# Autodesk Inventor assembly: ensamblaje jeringa
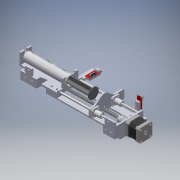
[picture p0: Inventor's stored thumbnail of the model, 180x180]
Saved by Autodesk Inventor 2019 (Build 230136000, 136)
## iProperties
Created: 2019-09-29
Part Number: ensamblaje jeringa
Document SubType Name: Assembly
Designer: dbrau
Author: dbrau
## Documents named in this file (13)
- D:\U\Semestre III mecánica\seminario\ensamblaje jeringa.iam
- D:\U\Semestre III mecánica\seminario\User Library-SYRINGE, MONOJECT, 60cc.ipt
- D:\U\Semestre III mecánica\seminario\sujeta_jeringa.ipt
- D:\U\Semestre III mecánica\seminario\NEMA 17 with T5 Pulley.iam
- D:\U\Semestre III mecánica\seminario\Acople flexible de aluminio (5mm a 8mm) Cimech 3D.ipt
- D:\U\Semestre III mecánica\seminario\Husillo Tr8x8 (p2) x 200mm real.ipt
- D:\U\Semestre III mecánica\seminario\LMK8UU.ipt
- D:\U\Semestre III mecánica\seminario\Tuerca Tr8x8 Cimech 3D.ipt
- D:\U\Semestre III mecánica\seminario\empuja_jeringa.ipt
- D:\U\Semestre III mecánica\seminario\sop_step_jeringa.ipt
- D:\U\Semestre III mecánica\seminario\eje_jeringa.ipt
- D:\U\Semestre III mecánica\seminario\union_jeringa.ipt
- D:\U\Semestre III mecánica\seminario\Endstop mecânico - Chave fim de curso.ipt
## Components (16 placed, 12 different names)
1. User Library-SYRINGE, MONOJECT, 60cc:1 — Insert:1, Flush:1
2. sujeta_jeringa:1 — Insert:1, Flush:1, Flush:2, Insert:14, Insert:15, Insert:20, Insert:21, Mate:3, Insert:22, Flush:3, Mate:4
3. NEMA 17 with T5 Pulley:1 [sub-assembly] — Insert:2, Insert:11, Insert:12
4. Acople flexible de aluminio (5mm a 8mm) Cimech 3D:1 — Insert:2, Insert:3
5. Husillo Tr8x8 (p2) x 200mm real:1 — Insert:3
6. LMK8UU:1 — Insert:7, Insert:8
7. LMK8UU:2 — Insert:9, Insert:10
8. Tuerca Tr8x8 Cimech 3D:1 — Insert:5, Insert:6
9. empuja_jeringa:1 — Insert:5, Insert:6, Insert:7, Insert:8, Insert:9, Insert:10, Flush:2, Mate:1, Insert:22, Flush:4
10. sop_step_jeringa:1 — Insert:11, Insert:12, Insert:16, Insert:17, Insert:18, Insert:19, Mate:5, Flush:5
11. eje_jeringa:1 — Insert:14
12. eje_jeringa:2 — Insert:15
13. union_jeringa:1 — Insert:16, Insert:17, Insert:20, Mate:1
14. union_jeringa:2 — Insert:18, Insert:19, Insert:21
15. Endstop mecânico - Chave fim de curso:1 — Mate:5, Flush:4, Flush:5
16. Endstop mecânico - Chave fim de curso:2 — Mate:3, Flush:3, Mate:4
## Relationships (29: Insert 20, Flush 5, Mate 4)
- Insert:1: User Library-SYRINGE, MONOJECT, 60cc:1 ↔ sujeta_jeringa:1
- Flush:1: User Library-SYRINGE, MONOJECT, 60cc:1 ↔ sujeta_jeringa:1
- Insert:2 (-12 mm): NEMA 17 with T5 Pulley:1 ↔ Acople flexible de aluminio (5mm a 8mm) Cimech 3D:1
- Insert:3 (-11 mm): Acople flexible de aluminio (5mm a 8mm) Cimech 3D:1 ↔ Husillo Tr8x8 (p2) x 200mm real:1
- Insert:5: Tuerca Tr8x8 Cimech 3D:1 ↔ empuja_jeringa:1
- Insert:6: Tuerca Tr8x8 Cimech 3D:1 ↔ empuja_jeringa:1
- Insert:7: LMK8UU:1 ↔ empuja_jeringa:1
- Insert:8: LMK8UU:1 ↔ empuja_jeringa:1
- Insert:9: LMK8UU:2 ↔ empuja_jeringa:1
- Insert:10: LMK8UU:2 ↔ empuja_jeringa:1
- Flush:2 (8.4 mm): sujeta_jeringa:1 ↔ empuja_jeringa:1
- Insert:11: NEMA 17 with T5 Pulley:1 ↔ sop_step_jeringa:1
- Insert:12: NEMA 17 with T5 Pulley:1 ↔ sop_step_jeringa:1
- Insert:14: sujeta_jeringa:1 ↔ eje_jeringa:1
- Insert:15: sujeta_jeringa:1 ↔ eje_jeringa:2
- Insert:16: sop_step_jeringa:1 ↔ union_jeringa:1
- Insert:17: sop_step_jeringa:1 ↔ union_jeringa:1
- Insert:18: sop_step_jeringa:1 ↔ union_jeringa:2
- Insert:19: sop_step_jeringa:1 ↔ union_jeringa:2
- Insert:20: sujeta_jeringa:1 ↔ union_jeringa:1
- Insert:21: sujeta_jeringa:1 ↔ union_jeringa:2
- Mate:1 (1.2 mm): empuja_jeringa:1 ↔ union_jeringa:1
- Mate:3 (25 mm): sujeta_jeringa:1 ↔ Endstop mecânico - Chave fim de curso:2
- Insert:22 (100 mm): sujeta_jeringa:1 ↔ empuja_jeringa:1
- Flush:3: sujeta_jeringa:1 ↔ Endstop mecânico - Chave fim de curso:2
- Mate:4: sujeta_jeringa:1 ↔ Endstop mecânico - Chave fim de curso:2
- Mate:5: sop_step_jeringa:1 ↔ Endstop mecânico - Chave fim de curso:1
- Flush:4: empuja_jeringa:1 ↔ Endstop mecânico - Chave fim de curso:1
- Flush:5: sop_step_jeringa:1 ↔ Endstop mecânico - Chave fim de curso:1
